# Autodesk Inventor assembly: ball joint
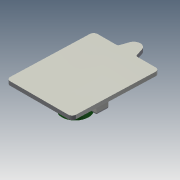
[picture p0: Inventor's stored thumbnail of the model, 180x180]
Saved by Autodesk Inventor 2015 (Build 190159000, 159)
## iProperties
Created: 2017-05-31
Part Number: ball joint
Document SubType Name: Assembly
Designer: gatew
Author: gatew
## Documents named in this file (3)
- C:\Users\gatew\Desktop\특허\ball joint.iam
- C:\Users\gatew\Desktop\특허\ball socket.ipt
- C:\Users\gatew\Desktop\특허\ball.ipt
## Components (3 placed, 2 different names)
1. ball socket:1 — 메이트:1, 메이트:2, 볼:1
2. ball socket:2 — 메이트:1, 메이트:2, 각도:1
3. ball:1 — 볼:1, 각도:1
## Relationships (4: Mate 2, BallJoint 1, Angle 1)
- 메이트:1 [Mate]: ball socket:1 ↔ ball socket:2
- 메이트:2 [Mate]: ball socket:1 ↔ ball socket:2
- 볼:1 [BallJoint]: ball socket:1 ↔ ball:1
- 각도:1 [Angle] (0 deg): ball socket:2 ↔ ball:1
